# Autodesk Inventor assembly: UpperArmRight
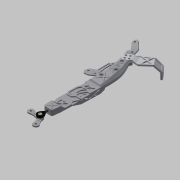
[picture p0: Inventor's stored thumbnail of the model, 180x180]
Saved by Autodesk Inventor 2015 SP1 (Build 190203100, 203)
## iProperties
Created: 2016-10-02
Part Number: UpperArmRight
Document SubType Name: Assembly
Designer: Val
Author: Val
## Documents named in this file (7)
- C:\Users\Val\Desktop\ExoGit\elysium-max-exoskeleton\src\Assemblies\UpperArmRight.iam
- C:\Users\Val\Desktop\ExoGit\elysium-max-exoskeleton\src\UpperArmRight.ipt
- C:\Users\Val\Desktop\ExoGit\elysium-max-exoskeleton\src\UpperArmShoulderRight.ipt
- C:\Users\Val\Desktop\ExoGit\elysium-max-exoskeleton\src\ElbowSubConnectorRight.ipt
- C:\Users\Val\Desktop\ExoGit\elysium-max-exoskeleton\src\UpperArmTricepRight.ipt
- C:\Users\Val\Desktop\ExoGit\elysium-max-exoskeleton\src\UpperArmConnectorRight.ipt
- C:\Users\Val\Desktop\ExoGit\elysium-max-exoskeleton\src\External\Bearing.iam
## Components (6 placed, 6 different names)
1. UpperArmRight:1 — Mate:1, Mate:2, Mate:3, Mate:4, Mate:5, Mate:6, Mate:7, Mate:8, Angle:1, Mate:9, Flush:1
2. UpperArmShoulderRight:1 — Mate:1, Mate:2, Mate:3
3. ElbowSubConnectorRight:1 — Mate:10, Mate:11
4. UpperArmTricepRight:1 — Mate:6, Mate:7, Mate:8
5. UpperArmTwistConnectorRight:1 — Mate:4, Mate:5
6. Bearing:1 [sub-assembly] — Angle:1, Mate:9, Mate:10, Mate:11, Flush:1
## Relationships (13: Mate 11, Angle 1, Flush 1)
- Mate:1: UpperArmRight:1 ↔ UpperArmShoulderRight:1
- Mate:2: UpperArmRight:1 ↔ UpperArmShoulderRight:1
- Mate:3: UpperArmRight:1 ↔ UpperArmShoulderRight:1
- Mate:4: UpperArmRight:1 ↔ UpperArmTwistConnectorRight:1
- Mate:5: UpperArmRight:1 ↔ UpperArmTwistConnectorRight:1
- Mate:6: UpperArmRight:1 ↔ UpperArmTricepRight:1
- Mate:7: UpperArmRight:1 ↔ UpperArmTricepRight:1
- Mate:8: UpperArmRight:1 ↔ UpperArmTricepRight:1
- Angle:1 (0 deg): UpperArmRight:1 ↔ Bearing:1
- Mate:9: UpperArmRight:1 ↔ Bearing:1
- Mate:10: ElbowSubConnectorRight:1 ↔ Bearing:1
- Mate:11: ElbowSubConnectorRight:1 ↔ Bearing:1
- Flush:1 (20 mm): UpperArmRight:1 ↔ Bearing:1
